# Autodesk Inventor assembly: ARm Gearbox
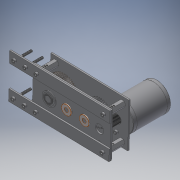
[picture p0: Inventor's stored thumbnail of the model, 180x180]
Saved by Autodesk Inventor 2018 (Build 220112000, 112)
## iProperties
Created: 2019-01-16
Part Number: ARm Gearbox
Document SubType Name: Assembly
Designer: Gabriel
Author: Gabriel
## Documents named in this file (22)
- C:\Users\s-4009421\Downloads\2019CAD-master (3)\2019CAD-master\New ARm Box\ARm Gearbox.iam
- C:\Users\s-4009421\Downloads\2019CAD-master (3)\2019CAD-master\New ARm Box\0_500_ID_x_1_125_OD_x_0_313_WD_Flanged_Bearing_217-2731.ipt
- C:\Users\s-4009421\Downloads\2019CAD-master (3)\2019CAD-master\New ARm Box\0.5in Hex Shaft.ipt
- C:\Users\s-4009421\Downloads\2019CAD-master (3)\2019CAD-master\New ARm Box\am-0150 Toughbox Large Output Gear.ipt
- C:\Users\s-4009421\Downloads\2019CAD-master (3)\2019CAD-master\New ARm Box\Mini_CIM_Motor_217-3371.ipt
- C:\Users\s-4009421\Downloads\2019CAD-master (3)\2019CAD-master\New ARm Box\ARm Gearbox Plate.ipt
- C:\Users\s-4009421\Downloads\2019CAD-master (3)\2019CAD-master\New ARm Box\1_16_Acetal_Spacer_-_1_2_Hex_217-3257.ipt
- C:\Users\s-4009421\Downloads\2019CAD-master (3)\2019CAD-master\New ARm Box\3_8in Hex Shaft.ipt
- C:\Users\s-4009421\Downloads\2019CAD-master (3)\2019CAD-master\New ARm Box\10T_Steel_Spur_Gear_20_DP_12T_Center_Distance_CIM_Motor_217-6334.ipt
- C:\Users\s-4009421\Downloads\2019CAD-master (3)\2019CAD-master\New ARm Box\am-0143 50 Tooth 20 dp Aluminum Gear 375 Hex.ipt
- C:\Users\s-4009421\Downloads\2019CAD-master (3)\2019CAD-master\New ARm Box\am-0151 14T 20dp 375hex.ipt
- C:\Users\s-4009421\Downloads\2019CAD-master (3)\2019CAD-master\New ARm Box\1_16_Acetal_Spacer_-_3_8_Hex_217-3258.ipt
- C:\Users\s-4009421\Downloads\2019CAD-master (3)\2019CAD-master\New ARm Box\40t_Aluminum_Spur_Gear_20_DP_3_8_Hex_Bore_217-2707.ipt
- C:\Users\s-4009421\Downloads\2019CAD-master (3)\2019CAD-master\New ARm Box\am-0028 00.375'' id Flanged, Shielded Ball Bearing (FR6ZZ).ipt
- C:\Users\s-4009421\Downloads\2019CAD-master (3)\2019CAD-master\New ARm Box\92196A271_18-8 STAINLESS STEEL SOCKET HEAD CAP SCREW.ipt
- C:\Users\s-4009421\Downloads\2019CAD-master (3)\2019CAD-master\New ARm Box\am-3621 - S25-18HA-500H.ipt
- C:\Users\s-4009421\Downloads\2019CAD-master (3)\2019CAD-master\New ARm Box\#10 Washer.ipt
- C:\Users\s-4009421\Downloads\2019CAD-master (3)\2019CAD-master\New ARm Box\Gearbox Mounting Gusset.ipt
- C:\Users\s-4009421\Downloads\2019CAD-master (3)\2019CAD-master\New ARm Box\1.5in 92196A251_18-8 STAINLESS STEEL SOCKET HEAD CAP SCREW.ipt
- C:\Users\s-4009421\Downloads\2019CAD-master (3)\2019CAD-master\New ARm Box\Churro For ARm Gearbox.ipt
- C:\Users\s-4009421\Downloads\2019CAD-master (3)\2019CAD-master\New ARm Box\.75in 92196A245_18-8 STAINLESS STEEL SOCKET HEAD CAP SCREW.ipt
- C:\Users\s-4009421\Downloads\.5 in spacer.ipt
## Components (55 placed, 21 different names)
1. 0.5in Hex Shaft:5 — Mate:345, Mate:346, Mate:347, Mate:348, Mate:349, Mate:350, Mate:351, Mate:386, Mate:387, Rotation:1, Mate:437, Mate:438, Mate:568, Mate:569, Mate:571, Mate:572, Mate:579
2. Mini_CIM_Motor_217-3371:5 — Mate:431, Mate:432, Mate:433, Mate:434, Mate:435, Mate:436
3. am-0150 Toughbox Large Output Gear:8 — Mate:345, Mate:346, Mate:347, Mate:352
4. 1_16_Acetal_Spacer_-_1_2_Hex_217-3257:4 — Mate:348, Mate:349, Mate:352, Mate:353
5. 1_16_Acetal_Spacer_-_1_2_Hex_217-3257:6 — Mate:350, Mate:351, Mate:353, Mate:354
6. 3_8in Hex Shaft:5 — Mate:313, Mate:314, Mate:315, Mate:316, Mate:317, Mate:318, Mate:321, Mate:322, Mate:357, Mate:358, Mate:411, Flush:2, Mate:425, Rotation:2
7. am-0151 14T 20dp 375hex:1 — Mate:325, Mate:326, Mate:331, Mate:335
8. am-0151 14T 20dp 375hex:3 — Mate:315, Mate:316, Mate:320, Mate:359
9. am-0143 50 Tooth 20 dp Aluminum Gear 375 Hex:5 — Mate:327, Mate:328, Mate:332, Mate:339
10. 10T_Steel_Spur_Gear_20_DP_12T_Center_Distance_CIM_Motor_217-6334:6 — Mate:434, Mate:435, Mate:436
11. 1_16_Acetal_Spacer_-_3_8_Hex_217-3258:2 — Mate:337, Mate:338, Mate:339
12. 1_16_Acetal_Spacer_-_3_8_Hex_217-3258:3 — Mate:333, Mate:334, Mate:335, Mate:422
13. 1_16_Acetal_Spacer_-_3_8_Hex_217-3258:5 — Mate:321, Mate:322, Mate:323, Mate:423
14. 1_16_Acetal_Spacer_-_3_8_Hex_217-3258:6 — Mate:317, Mate:318, Mate:319, Mate:320
15. 40t_Aluminum_Spur_Gear_20_DP_3_8_Hex_Bore_217-2707:1 — Mate:313, Mate:314, Mate:319, Mate:323
16. 3_8in Hex Shaft:10 — Mate:325, Mate:326, Mate:327, Mate:328, Mate:329, Mate:330, Mate:333, Mate:334, Mate:337, Mate:338, Mate:412, Flush:1, Mate:424, Mate:426, Rotation:3
17. ARm Gearbox Plate:5 — Mate:341, Mate:344, Mate:413, Mate:414, Mate:415, Mate:416, Mate:451, Mate:452, Mate:453, Mate:454, Mate:455, Mate:456, Mate:537, Mate:539, Mate:541, Mate:543
18. ARm Gearbox Plate:6 — Mate:342, Mate:343, Mate:360, Mate:361, Mate:362, Mate:363, Mate:407, Mate:408, Mate:409, Mate:410, Mate:419, Mate:421, Rotation:1, Mate:544, Mate:546, Mate:547, Mate:548, Mate:549, Mate:553, Mate:554, Mate:555
19. 1_16_Acetal_Spacer_-_3_8_Hex_217-3258:8 — Mate:357, Mate:358, Mate:359
20. 1_16_Acetal_Spacer_-_3_8_Hex_217-3258:10 — Mate:329, Mate:330, Mate:331, Mate:332
21. 0_500_ID_x_1_125_OD_x_0_313_WD_Flanged_Bearing_217-2731:9 — Mate:341, Mate:344, Mate:439
22. 0_500_ID_x_1_125_OD_x_0_313_WD_Flanged_Bearing_217-2731:10 — Mate:342, Mate:343, Mate:354, Mate:576
23. 92196A271_18-8 STAINLESS STEEL SOCKET HEAD CAP SCREW:1 — Mate:361, Mate:363, Mate:420, Mate:429, Mate:431
24. 92196A271_18-8 STAINLESS STEEL SOCKET HEAD CAP SCREW:2 — Mate:360, Mate:362, Mate:417, Mate:427, Mate:432
25. am-0028 00.375'' id Flanged, Shielded Ball Bearing (FR6ZZ):3 — Mate:414, Mate:416, Mate:425, Rotation:2
26. am-0028 00.375'' id Flanged, Shielded Ball Bearing (FR6ZZ):4 — Mate:413, Mate:415, Mate:424, Mate:426, Rotation:3
27. am-3621 - S25-18HA-500H:1 — Mate:386, Mate:387, Mate:570, Mate:575, Mate:577
28. am-0028 00.375'' id Flanged, Shielded Ball Bearing (FR6ZZ):5 — Mate:409, Mate:410, Mate:411, Flush:2, Mate:423
29. am-0028 00.375'' id Flanged, Shielded Ball Bearing (FR6ZZ):6 — Mate:407, Mate:408, Mate:412, Flush:1, Mate:422
30. #10 Washer:1 — Mate:417, Mate:419, Mate:428
31. #10 Washer:2 — Mate:420, Mate:421, Mate:430
32. #10 Washer:3 — Mate:427, Mate:428, Mate:433
33. #10 Washer:4 — Mate:429, Mate:430
34. 1_16_Acetal_Spacer_-_1_2_Hex_217-3257:9 — Mate:437, Mate:438, Mate:439, Mate:579
35. Gearbox Mounting Gusset:1 — Mate:451, Mate:452, Mate:453, Mate:528, Mate:529, Mate:532, Mate:535, Mate:558, Mate:559, Mate:560, Mate:561
36. Gearbox Mounting Gusset:2 — Mate:454, Mate:455, Mate:456, Mate:530, Mate:531, Mate:533, Mate:534, Mate:562, Mate:563, Mate:564, Mate:565
37. Churro For ARm Gearbox:1 — Mate:540, Mate:541, Mate:545
38. Churro For ARm Gearbox:2 — Mate:538, Mate:539, Mate:550
39. Churro For ARm Gearbox:3 — Mate:542, Mate:543, Mate:552
40. Churro For ARm Gearbox:4 — Mate:536, Mate:537, Mate:551
41. .75in 92196A245_18-8 STAINLESS STEEL SOCKET HEAD CAP SCREW:1 — Mate:531, Mate:534, Mate:542
42. .75in 92196A245_18-8 STAINLESS STEEL SOCKET HEAD CAP SCREW:2 — Mate:528, Mate:529, Mate:536
43. .75in 92196A245_18-8 STAINLESS STEEL SOCKET HEAD CAP SCREW:3 — Mate:532, Mate:535, Mate:538
44. .75in 92196A245_18-8 STAINLESS STEEL SOCKET HEAD CAP SCREW:4 — Mate:530, Mate:533, Mate:540
45. .75in 92196A245_18-8 STAINLESS STEEL SOCKET HEAD CAP SCREW:5 — Mate:549, Mate:552, Mate:555
46. .75in 92196A245_18-8 STAINLESS STEEL SOCKET HEAD CAP SCREW:6 — Mate:547, Mate:550, Mate:553
47. .75in 92196A245_18-8 STAINLESS STEEL SOCKET HEAD CAP SCREW:7 — Mate:548, Mate:551, Mate:554
48. .75in 92196A245_18-8 STAINLESS STEEL SOCKET HEAD CAP SCREW:8 — Mate:544, Mate:545, Mate:546
49. 1.5in 92196A251_18-8 STAINLESS STEEL SOCKET HEAD CAP SCREW:3 — Mate:558, Mate:559
50. 1.5in 92196A251_18-8 STAINLESS STEEL SOCKET HEAD CAP SCREW:6 — Mate:563, Mate:565
51. 1.5in 92196A251_18-8 STAINLESS STEEL SOCKET HEAD CAP SCREW:7 — Mate:562, Mate:564
52. 1.5in 92196A251_18-8 STAINLESS STEEL SOCKET HEAD CAP SCREW:8 — Mate:560, Mate:561
53. 1_16_Acetal_Spacer_-_1_2_Hex_217-3257:10 — Mate:568, Mate:569, Mate:570, Mate:573, Mate:574
54. 1_16_Acetal_Spacer_-_1_2_Hex_217-3257:11 — Mate:571, Mate:572, Mate:573, Mate:574
55. .5 in spacer:1 — Mate:575, Mate:576, Mate:577
## Relationships (138: Mate 133, RelateRotation 3, Flush 2)
- Mate:313: 3_8in Hex Shaft:5 ↔ 40t_Aluminum_Spur_Gear_20_DP_3_8_Hex_Bore_217-2707:1
- Mate:314: 3_8in Hex Shaft:5 ↔ 40t_Aluminum_Spur_Gear_20_DP_3_8_Hex_Bore_217-2707:1
- Mate:315: 3_8in Hex Shaft:5 ↔ am-0151 14T 20dp 375hex:3
- Mate:316: 3_8in Hex Shaft:5 ↔ am-0151 14T 20dp 375hex:3
- Mate:317: 3_8in Hex Shaft:5 ↔ 1_16_Acetal_Spacer_-_3_8_Hex_217-3258:6
- Mate:318: 3_8in Hex Shaft:5 ↔ 1_16_Acetal_Spacer_-_3_8_Hex_217-3258:6
- Mate:319: 1_16_Acetal_Spacer_-_3_8_Hex_217-3258:6 ↔ 40t_Aluminum_Spur_Gear_20_DP_3_8_Hex_Bore_217-2707:1
- Mate:320: am-0151 14T 20dp 375hex:3 ↔ 1_16_Acetal_Spacer_-_3_8_Hex_217-3258:6
- Mate:321: 3_8in Hex Shaft:5 ↔ 1_16_Acetal_Spacer_-_3_8_Hex_217-3258:5
- Mate:322: 3_8in Hex Shaft:5 ↔ 1_16_Acetal_Spacer_-_3_8_Hex_217-3258:5
- Mate:323: 1_16_Acetal_Spacer_-_3_8_Hex_217-3258:5 ↔ 40t_Aluminum_Spur_Gear_20_DP_3_8_Hex_Bore_217-2707:1
- Mate:325: am-0151 14T 20dp 375hex:1 ↔ 3_8in Hex Shaft:10
- Mate:326: am-0151 14T 20dp 375hex:1 ↔ 3_8in Hex Shaft:10
- Mate:327: am-0143 50 Tooth 20 dp Aluminum Gear 375 Hex:5 ↔ 3_8in Hex Shaft:10
- Mate:328: am-0143 50 Tooth 20 dp Aluminum Gear 375 Hex:5 ↔ 3_8in Hex Shaft:10
- Mate:329: 3_8in Hex Shaft:10 ↔ 1_16_Acetal_Spacer_-_3_8_Hex_217-3258:10
- Mate:330: 3_8in Hex Shaft:10 ↔ 1_16_Acetal_Spacer_-_3_8_Hex_217-3258:10
- Mate:331: am-0151 14T 20dp 375hex:1 ↔ 1_16_Acetal_Spacer_-_3_8_Hex_217-3258:10
- Mate:332: am-0143 50 Tooth 20 dp Aluminum Gear 375 Hex:5 ↔ 1_16_Acetal_Spacer_-_3_8_Hex_217-3258:10
- Mate:333: 1_16_Acetal_Spacer_-_3_8_Hex_217-3258:3 ↔ 3_8in Hex Shaft:10
- Mate:334: 1_16_Acetal_Spacer_-_3_8_Hex_217-3258:3 ↔ 3_8in Hex Shaft:10
- Mate:335: am-0151 14T 20dp 375hex:1 ↔ 1_16_Acetal_Spacer_-_3_8_Hex_217-3258:3
- Mate:337: 1_16_Acetal_Spacer_-_3_8_Hex_217-3258:2 ↔ 3_8in Hex Shaft:10
- Mate:338: 1_16_Acetal_Spacer_-_3_8_Hex_217-3258:2 ↔ 3_8in Hex Shaft:10
- Mate:339: am-0143 50 Tooth 20 dp Aluminum Gear 375 Hex:5 ↔ 1_16_Acetal_Spacer_-_3_8_Hex_217-3258:2
- Mate:341: ARm Gearbox Plate:5 ↔ 0_500_ID_x_1_125_OD_x_0_313_WD_Flanged_Bearing_217-2731:9
- Mate:342: ARm Gearbox Plate:6 ↔ 0_500_ID_x_1_125_OD_x_0_313_WD_Flanged_Bearing_217-2731:10
- Mate:343: ARm Gearbox Plate:6 ↔ 0_500_ID_x_1_125_OD_x_0_313_WD_Flanged_Bearing_217-2731:10
- Mate:344: ARm Gearbox Plate:5 ↔ 0_500_ID_x_1_125_OD_x_0_313_WD_Flanged_Bearing_217-2731:9
- Mate:345: 0.5in Hex Shaft:5 ↔ am-0150 Toughbox Large Output Gear:8
- Mate:346: 0.5in Hex Shaft:5 ↔ am-0150 Toughbox Large Output Gear:8
- Mate:347: 0.5in Hex Shaft:5 ↔ am-0150 Toughbox Large Output Gear:8
- Mate:348: 0.5in Hex Shaft:5 ↔ 1_16_Acetal_Spacer_-_1_2_Hex_217-3257:4
- Mate:349: 0.5in Hex Shaft:5 ↔ 1_16_Acetal_Spacer_-_1_2_Hex_217-3257:4
- Mate:350: 0.5in Hex Shaft:5 ↔ 1_16_Acetal_Spacer_-_1_2_Hex_217-3257:6
- Mate:351: 0.5in Hex Shaft:5 ↔ 1_16_Acetal_Spacer_-_1_2_Hex_217-3257:6
- Mate:352: am-0150 Toughbox Large Output Gear:8 ↔ 1_16_Acetal_Spacer_-_1_2_Hex_217-3257:4
- Mate:353: 1_16_Acetal_Spacer_-_1_2_Hex_217-3257:4 ↔ 1_16_Acetal_Spacer_-_1_2_Hex_217-3257:6
- Mate:354: 1_16_Acetal_Spacer_-_1_2_Hex_217-3257:6 ↔ 0_500_ID_x_1_125_OD_x_0_313_WD_Flanged_Bearing_217-2731:10
- Mate:357: 3_8in Hex Shaft:5 ↔ 1_16_Acetal_Spacer_-_3_8_Hex_217-3258:8
- Mate:358: 3_8in Hex Shaft:5 ↔ 1_16_Acetal_Spacer_-_3_8_Hex_217-3258:8
- Mate:359: am-0151 14T 20dp 375hex:3 ↔ 1_16_Acetal_Spacer_-_3_8_Hex_217-3258:8
- Mate:360: ARm Gearbox Plate:6 ↔ 92196A271_18-8 STAINLESS STEEL SOCKET HEAD CAP SCREW:2
- Mate:361: ARm Gearbox Plate:6 ↔ 92196A271_18-8 STAINLESS STEEL SOCKET HEAD CAP SCREW:1
- Mate:362: ARm Gearbox Plate:6 ↔ 92196A271_18-8 STAINLESS STEEL SOCKET HEAD CAP SCREW:2
- Mate:363: ARm Gearbox Plate:6 ↔ 92196A271_18-8 STAINLESS STEEL SOCKET HEAD CAP SCREW:1
- Mate:386: 0.5in Hex Shaft:5 ↔ am-3621 - S25-18HA-500H:1
- Mate:387: 0.5in Hex Shaft:5 ↔ am-3621 - S25-18HA-500H:1
- Mate:407: ARm Gearbox Plate:6 ↔ am-0028 00.375'' id Flanged, Shielded Ball Bearing (FR6ZZ):6
- Mate:408: ARm Gearbox Plate:6 ↔ am-0028 00.375'' id Flanged, Shielded Ball Bearing (FR6ZZ):6
- Mate:409: ARm Gearbox Plate:6 ↔ am-0028 00.375'' id Flanged, Shielded Ball Bearing (FR6ZZ):5
- Mate:410: ARm Gearbox Plate:6 ↔ am-0028 00.375'' id Flanged, Shielded Ball Bearing (FR6ZZ):5
- Mate:411: 3_8in Hex Shaft:5 ↔ am-0028 00.375'' id Flanged, Shielded Ball Bearing (FR6ZZ):5
- Mate:412: 3_8in Hex Shaft:10 ↔ am-0028 00.375'' id Flanged, Shielded Ball Bearing (FR6ZZ):6
- Mate:413: ARm Gearbox Plate:5 ↔ am-0028 00.375'' id Flanged, Shielded Ball Bearing (FR6ZZ):4
- Mate:414: ARm Gearbox Plate:5 ↔ am-0028 00.375'' id Flanged, Shielded Ball Bearing (FR6ZZ):3
- Mate:415: ARm Gearbox Plate:5 ↔ am-0028 00.375'' id Flanged, Shielded Ball Bearing (FR6ZZ):4
- Mate:416: ARm Gearbox Plate:5 ↔ am-0028 00.375'' id Flanged, Shielded Ball Bearing (FR6ZZ):3
- Mate:417: 92196A271_18-8 STAINLESS STEEL SOCKET HEAD CAP SCREW:2 ↔ #10 Washer:1
- Mate:419: ARm Gearbox Plate:6 ↔ #10 Washer:1
- Mate:420: 92196A271_18-8 STAINLESS STEEL SOCKET HEAD CAP SCREW:1 ↔ #10 Washer:2
- Mate:421: ARm Gearbox Plate:6 ↔ #10 Washer:2
- Flush:1: 3_8in Hex Shaft:10 ↔ am-0028 00.375'' id Flanged, Shielded Ball Bearing (FR6ZZ):6
- Flush:2: 3_8in Hex Shaft:5 ↔ am-0028 00.375'' id Flanged, Shielded Ball Bearing (FR6ZZ):5
- Rotation:1 [RelateRotation] (1 ul): 0.5in Hex Shaft:5 ↔ ARm Gearbox Plate:6
- Mate:422: 1_16_Acetal_Spacer_-_3_8_Hex_217-3258:3 ↔ am-0028 00.375'' id Flanged, Shielded Ball Bearing (FR6ZZ):6
- Mate:423: 1_16_Acetal_Spacer_-_3_8_Hex_217-3258:5 ↔ am-0028 00.375'' id Flanged, Shielded Ball Bearing (FR6ZZ):5
- Mate:424: 3_8in Hex Shaft:10 ↔ am-0028 00.375'' id Flanged, Shielded Ball Bearing (FR6ZZ):4
- Mate:425: 3_8in Hex Shaft:5 ↔ am-0028 00.375'' id Flanged, Shielded Ball Bearing (FR6ZZ):3
- Mate:426: 3_8in Hex Shaft:10 ↔ am-0028 00.375'' id Flanged, Shielded Ball Bearing (FR6ZZ):4
- Rotation:2 [RelateRotation] (1 ul): 3_8in Hex Shaft:5 ↔ am-0028 00.375'' id Flanged, Shielded Ball Bearing (FR6ZZ):3
- Rotation:3 [RelateRotation] (1 ul): 3_8in Hex Shaft:10 ↔ am-0028 00.375'' id Flanged, Shielded Ball Bearing (FR6ZZ):4
- Mate:427: 92196A271_18-8 STAINLESS STEEL SOCKET HEAD CAP SCREW:2 ↔ #10 Washer:3
- Mate:428: #10 Washer:1 ↔ #10 Washer:3
- Mate:429: 92196A271_18-8 STAINLESS STEEL SOCKET HEAD CAP SCREW:1 ↔ #10 Washer:4
- Mate:430: #10 Washer:2 ↔ #10 Washer:4
- Mate:431: Mini_CIM_Motor_217-3371:5 ↔ 92196A271_18-8 STAINLESS STEEL SOCKET HEAD CAP SCREW:1
- Mate:432: Mini_CIM_Motor_217-3371:5 ↔ 92196A271_18-8 STAINLESS STEEL SOCKET HEAD CAP SCREW:2
- Mate:433: Mini_CIM_Motor_217-3371:5 ↔ #10 Washer:3
- Mate:434: Mini_CIM_Motor_217-3371:5 ↔ 10T_Steel_Spur_Gear_20_DP_12T_Center_Distance_CIM_Motor_217-6334:6
- Mate:435: Mini_CIM_Motor_217-3371:5 ↔ 10T_Steel_Spur_Gear_20_DP_12T_Center_Distance_CIM_Motor_217-6334:6
- Mate:436: Mini_CIM_Motor_217-3371:5 ↔ 10T_Steel_Spur_Gear_20_DP_12T_Center_Distance_CIM_Motor_217-6334:6
- Mate:437: 0.5in Hex Shaft:5 ↔ 1_16_Acetal_Spacer_-_1_2_Hex_217-3257:9
- Mate:438: 0.5in Hex Shaft:5 ↔ 1_16_Acetal_Spacer_-_1_2_Hex_217-3257:9
- Mate:439: 0_500_ID_x_1_125_OD_x_0_313_WD_Flanged_Bearing_217-2731:9 ↔ 1_16_Acetal_Spacer_-_1_2_Hex_217-3257:9
- Mate:451: ARm Gearbox Plate:5 ↔ Gearbox Mounting Gusset:1
- Mate:452: ARm Gearbox Plate:5 ↔ Gearbox Mounting Gusset:1
- Mate:453: ARm Gearbox Plate:5 ↔ Gearbox Mounting Gusset:1
- Mate:454: ARm Gearbox Plate:5 ↔ Gearbox Mounting Gusset:2
- Mate:455: ARm Gearbox Plate:5 ↔ Gearbox Mounting Gusset:2
- Mate:456: ARm Gearbox Plate:5 ↔ Gearbox Mounting Gusset:2
- Mate:528: Gearbox Mounting Gusset:1 ↔ .75in 92196A245_18-8 STAINLESS STEEL SOCKET HEAD CAP SCREW:2
- Mate:529: Gearbox Mounting Gusset:1 ↔ .75in 92196A245_18-8 STAINLESS STEEL SOCKET HEAD CAP SCREW:2
- Mate:530: Gearbox Mounting Gusset:2 ↔ .75in 92196A245_18-8 STAINLESS STEEL SOCKET HEAD CAP SCREW:4
- Mate:531: Gearbox Mounting Gusset:2 ↔ .75in 92196A245_18-8 STAINLESS STEEL SOCKET HEAD CAP SCREW:1
- Mate:532: Gearbox Mounting Gusset:1 ↔ .75in 92196A245_18-8 STAINLESS STEEL SOCKET HEAD CAP SCREW:3
- Mate:533: Gearbox Mounting Gusset:2 ↔ .75in 92196A245_18-8 STAINLESS STEEL SOCKET HEAD CAP SCREW:4
- Mate:534: Gearbox Mounting Gusset:2 ↔ .75in 92196A245_18-8 STAINLESS STEEL SOCKET HEAD CAP SCREW:1
- Mate:535: Gearbox Mounting Gusset:1 ↔ .75in 92196A245_18-8 STAINLESS STEEL SOCKET HEAD CAP SCREW:3
- Mate:536: Churro For ARm Gearbox:4 ↔ .75in 92196A245_18-8 STAINLESS STEEL SOCKET HEAD CAP SCREW:2
- Mate:537: ARm Gearbox Plate:5 ↔ Churro For ARm Gearbox:4
- Mate:538: Churro For ARm Gearbox:2 ↔ .75in 92196A245_18-8 STAINLESS STEEL SOCKET HEAD CAP SCREW:3
- Mate:539: ARm Gearbox Plate:5 ↔ Churro For ARm Gearbox:2
- Mate:540: Churro For ARm Gearbox:1 ↔ .75in 92196A245_18-8 STAINLESS STEEL SOCKET HEAD CAP SCREW:4
- Mate:541: ARm Gearbox Plate:5 ↔ Churro For ARm Gearbox:1
- Mate:542: Churro For ARm Gearbox:3 ↔ .75in 92196A245_18-8 STAINLESS STEEL SOCKET HEAD CAP SCREW:1
- Mate:543: ARm Gearbox Plate:5 ↔ Churro For ARm Gearbox:3
- Mate:544: ARm Gearbox Plate:6 ↔ .75in 92196A245_18-8 STAINLESS STEEL SOCKET HEAD CAP SCREW:8
- Mate:545: Churro For ARm Gearbox:1 ↔ .75in 92196A245_18-8 STAINLESS STEEL SOCKET HEAD CAP SCREW:8
- Mate:546: ARm Gearbox Plate:6 ↔ .75in 92196A245_18-8 STAINLESS STEEL SOCKET HEAD CAP SCREW:8
- Mate:547: ARm Gearbox Plate:6 ↔ .75in 92196A245_18-8 STAINLESS STEEL SOCKET HEAD CAP SCREW:6
- Mate:548: ARm Gearbox Plate:6 ↔ .75in 92196A245_18-8 STAINLESS STEEL SOCKET HEAD CAP SCREW:7
- Mate:549: ARm Gearbox Plate:6 ↔ .75in 92196A245_18-8 STAINLESS STEEL SOCKET HEAD CAP SCREW:5
- Mate:550: Churro For ARm Gearbox:2 ↔ .75in 92196A245_18-8 STAINLESS STEEL SOCKET HEAD CAP SCREW:6
- Mate:551: Churro For ARm Gearbox:4 ↔ .75in 92196A245_18-8 STAINLESS STEEL SOCKET HEAD CAP SCREW:7
- Mate:552: Churro For ARm Gearbox:3 ↔ .75in 92196A245_18-8 STAINLESS STEEL SOCKET HEAD CAP SCREW:5
- Mate:553: ARm Gearbox Plate:6 ↔ .75in 92196A245_18-8 STAINLESS STEEL SOCKET HEAD CAP SCREW:6
- Mate:554: ARm Gearbox Plate:6 ↔ .75in 92196A245_18-8 STAINLESS STEEL SOCKET HEAD CAP SCREW:7
- Mate:555: ARm Gearbox Plate:6 ↔ .75in 92196A245_18-8 STAINLESS STEEL SOCKET HEAD CAP SCREW:5
- Mate:558: Gearbox Mounting Gusset:1 ↔ 1.5in 92196A251_18-8 STAINLESS STEEL SOCKET HEAD CAP SCREW:3
- Mate:559: Gearbox Mounting Gusset:1 ↔ 1.5in 92196A251_18-8 STAINLESS STEEL SOCKET HEAD CAP SCREW:3
- Mate:560: Gearbox Mounting Gusset:1 ↔ 1.5in 92196A251_18-8 STAINLESS STEEL SOCKET HEAD CAP SCREW:8
- Mate:561: Gearbox Mounting Gusset:1 ↔ 1.5in 92196A251_18-8 STAINLESS STEEL SOCKET HEAD CAP SCREW:8
- Mate:562: Gearbox Mounting Gusset:2 ↔ 1.5in 92196A251_18-8 STAINLESS STEEL SOCKET HEAD CAP SCREW:7
- Mate:563: Gearbox Mounting Gusset:2 ↔ 1.5in 92196A251_18-8 STAINLESS STEEL SOCKET HEAD CAP SCREW:6
- Mate:564: Gearbox Mounting Gusset:2 ↔ 1.5in 92196A251_18-8 STAINLESS STEEL SOCKET HEAD CAP SCREW:7
- Mate:565: Gearbox Mounting Gusset:2 ↔ 1.5in 92196A251_18-8 STAINLESS STEEL SOCKET HEAD CAP SCREW:6
- Mate:568: 0.5in Hex Shaft:5 ↔ 1_16_Acetal_Spacer_-_1_2_Hex_217-3257:10
- Mate:569: 0.5in Hex Shaft:5 ↔ 1_16_Acetal_Spacer_-_1_2_Hex_217-3257:10
- Mate:570: am-3621 - S25-18HA-500H:1 ↔ 1_16_Acetal_Spacer_-_1_2_Hex_217-3257:10
- Mate:571: 0.5in Hex Shaft:5 ↔ 1_16_Acetal_Spacer_-_1_2_Hex_217-3257:11
- Mate:572: 0.5in Hex Shaft:5 ↔ 1_16_Acetal_Spacer_-_1_2_Hex_217-3257:11
- Mate:573: 1_16_Acetal_Spacer_-_1_2_Hex_217-3257:10 ↔ 1_16_Acetal_Spacer_-_1_2_Hex_217-3257:11
- Mate:574: 1_16_Acetal_Spacer_-_1_2_Hex_217-3257:10 ↔ 1_16_Acetal_Spacer_-_1_2_Hex_217-3257:11
- Mate:575: am-3621 - S25-18HA-500H:1 ↔ .5 in spacer:1
- Mate:576: 0_500_ID_x_1_125_OD_x_0_313_WD_Flanged_Bearing_217-2731:10 ↔ .5 in spacer:1
- Mate:577: am-3621 - S25-18HA-500H:1 ↔ .5 in spacer:1
- Mate:579: 0.5in Hex Shaft:5 ↔ 1_16_Acetal_Spacer_-_1_2_Hex_217-3257:9
